# Autodesk Inventor assembly: Montagem dianteira
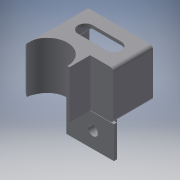
[picture p0: Inventor's stored thumbnail of the model, 180x180]
Saved by Autodesk Inventor 2019 (Build 230136000, 136)
## iProperties
Created: 2021-06-28
Part Number: Montagem dianteira
Material: Genérico
Document SubType Name: Assembly
Designer: SOU O MELHOR
Author: SOU O MELHOR
## Documents named in this file (3)
- F:\Lucas\BAJA\Inventor\Atividades\Nova fixação do acelerometro 2\Montagem dianteira.iam
- F:\Lucas\BAJA\Inventor\Atividades\Nova fixação do acelerometro 2\Caixa dianteira.ipt
- F:\Lucas\BAJA\Inventor\Atividades\Nova fixação do acelerometro 2\Fixador acelerometro dianteiro.ipt
## Components (2 placed, 2 different names)
1. Caixa dianteira:1 — Coincidência:1
2. Fixador acelerometro dianteiro:1 — Coincidência:1
## Relationships (1: Mate 1)
- Coincidência:1 [Mate]: Caixa dianteira:1 ↔ Fixador acelerometro dianteiro:1
